# Autodesk Inventor assembly: Conjuntocontenedor
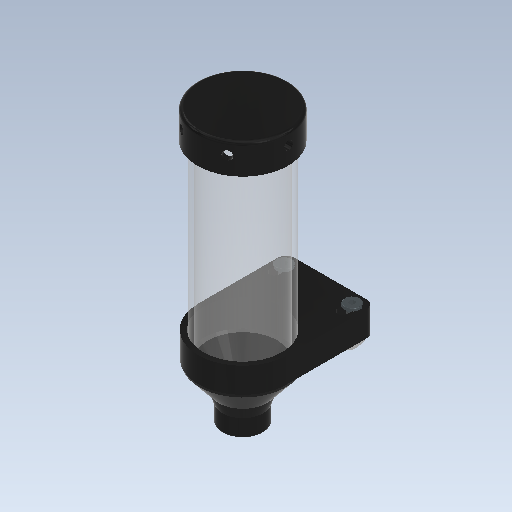
[picture p0: Inventor's stored thumbnail of the model, 512x512]
Saved by Autodesk Inventor 2020.2 (Build 242310000, 310)
## iProperties
Created: 2021-01-05
Part Number: Conjuntocontenedor
Document SubType Name: Assembly
Designer: JK
Author: JK
## Documents named in this file (6)
- C:\Users\JK\Documents\Inventor\BioMixer\DispensadorPolvo\Conjuntocontenedor.iam
- C:\Users\JK\Documents\Inventor\BioMixer\ContenedorPolvosyGlicerina.ipt
- C:\Users\JK\Documents\Inventor\BioMixer\Tapacontenedor.ipt
- C:\Users\JK\Documents\Inventor\BioMixer\DispensadorPolvo\BaseContenedorPolvos.ipt
- C:\Users\JK\Documents\Inventor\BioMixer\DispensadorPolvo\PernoM5x20Plano.ipt
- C:\Users\JK\Documents\Inventor\BioMixer\DispensadorPolvo\TuercaTM5Perfil2020.ipt
## Components (7 placed, 5 different names)
1. BaseContenedorPolvos:1 — Mate:5, Mate:6, Mate:7, Mate:8, Mate:9, Mate:12
2. ContenedorPolvosyGlicerina:1 — Mate:3, Mate:4, Mate:5, Mate:6
3. Tapacontenedor:1 — Mate:3, Mate:4
4. PernoM5x20Plano:1 — Mate:8, Flush:1, Mate:11
5. PernoM5x20Plano:2 — Mate:7, Flush:1, Mate:9, Mate:10
6. TuercaTM5Perfil2020:1 — Mate:11, Angle:1, Flush:2
7. TuercaTM5Perfil2020:2 — Mate:10, Angle:1, Mate:12, Flush:2
## Relationships (13: Mate 10, Flush 2, Angle 1)
- Mate:3: ContenedorPolvosyGlicerina:1 ↔ Tapacontenedor:1
- Mate:4: ContenedorPolvosyGlicerina:1 ↔ Tapacontenedor:1
- Mate:5: BaseContenedorPolvos:1 ↔ ContenedorPolvosyGlicerina:1
- Mate:6: BaseContenedorPolvos:1 ↔ ContenedorPolvosyGlicerina:1
- Mate:7: BaseContenedorPolvos:1 ↔ PernoM5x20Plano:2
- Mate:8: BaseContenedorPolvos:1 ↔ PernoM5x20Plano:1
- Flush:1: PernoM5x20Plano:1 ↔ PernoM5x20Plano:2
- Mate:9: BaseContenedorPolvos:1 ↔ PernoM5x20Plano:2
- Mate:10: PernoM5x20Plano:2 ↔ TuercaTM5Perfil2020:2
- Mate:11: PernoM5x20Plano:1 ↔ TuercaTM5Perfil2020:1
- Angle:1 (0 deg): TuercaTM5Perfil2020:1 ↔ TuercaTM5Perfil2020:2
- Mate:12 (0.5 mm): BaseContenedorPolvos:1 ↔ TuercaTM5Perfil2020:2
- Flush:2: TuercaTM5Perfil2020:1 ↔ TuercaTM5Perfil2020:2
